# Autodesk Inventor assembly: Segment_Staender_v1
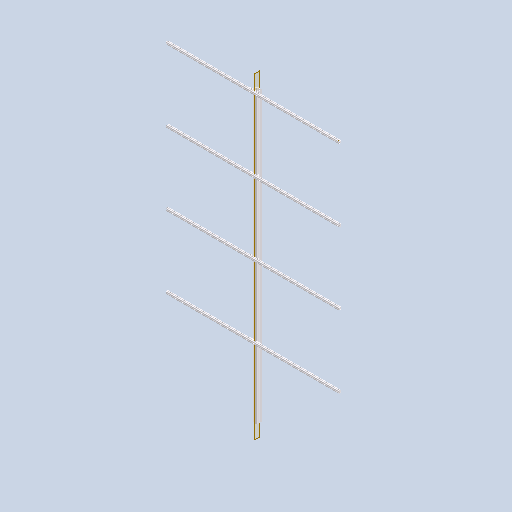
[picture p0: Inventor's stored thumbnail of the model, 512x512]
Saved by Autodesk Inventor 2025.1 (Build 291241000, 241)
## iProperties
Created: 2024-10-13
Part Number: Segment_Staender_v1
Document SubType Name: Assembly
Designer: Kai Altwicker
Author: Kai Altwicker
## Documents named in this file (5)
- C:\Users\tallA\Repos\VolumanXR\hardware-capture\cad\rig_v1\Segment_Staender_v1.iam
- C:\Users\tallA\Repos\VolumanXR\hardware-capture\cad\Library\Profil_5_40x40_2500\Profil_5_40x40_2500\Profil_5_40x40_2500.ipt
- C:\Users\tallA\Repos\VolumanXR\hardware-capture\cad\rig_v1\Profil_5_20x20_1500.ipt
- C:\Users\tallA\Repos\VolumanXR\hardware-capture\cad\Library\Winkelsatz_20x20_einfach\Winkelsatz_20x20_einfach\Winkelsatz_20x20_einfach.ipt
- C:\Users\tallA\Repos\VolumanXR\hardware-capture\cad\dimensions.xlsx
## Components (13 placed, 3 different names)
1. Profil_5_40x40_2500:1 — Passend:4, Fluchtend:7, Passend:5, Fluchtend:11, Passend:7
2. Winkelsatz_20x20_einfach:1 — Passend:5, Passend:6, Fluchtend:10, Fluchtend:12
3. Profil_5_20x20_1500:1 — Passend:4, Fluchtend:7, Passend:6, Fluchtend:10, Fluchtend:11, Passend:8, Passend:9, Passend:10
4. Winkelsatz_20x20_einfach:2 — Passend:7, Passend:8, Fluchtend:12
5. Winkelsatz_20x20_einfach:3
6. Profil_5_20x20_1500:2
7. Winkelsatz_20x20_einfach:4
8. Winkelsatz_20x20_einfach:5
9. Profil_5_20x20_1500:3
10. Winkelsatz_20x20_einfach:6
11. Winkelsatz_20x20_einfach:7
12. Profil_5_20x20_1500:4
13. Winkelsatz_20x20_einfach:8
## Component patterns: (4 elements, first: Winkelsatz_20x20_einfach:1 + Profil_5_20x20_1500:1 + Winkelsatz_20x20_einfach:2)
## Relationships (11: Mate 7, Flush 4)
- Passend:4 [Mate]: Profil_5_40x40_2500:1 ↔ Profil_5_20x20_1500:1
- Fluchtend:7 [Flush]: Profil_5_40x40_2500:1 ↔ Profil_5_20x20_1500:1
- Passend:5 [Mate]: Profil_5_40x40_2500:1 ↔ Winkelsatz_20x20_einfach:1
- Passend:6 [Mate]: Winkelsatz_20x20_einfach:1 ↔ Profil_5_20x20_1500:1
- Fluchtend:10 [Flush]: Winkelsatz_20x20_einfach:1 ↔ Profil_5_20x20_1500:1
- Fluchtend:11 [Flush] (-750 mm): Profil_5_40x40_2500:1 ↔ Profil_5_20x20_1500:1
- Passend:7 [Mate]: Profil_5_40x40_2500:1 ↔ Winkelsatz_20x20_einfach:2
- Passend:8 [Mate]: Profil_5_20x20_1500:1 ↔ Winkelsatz_20x20_einfach:2
- Fluchtend:12 [Flush]: Winkelsatz_20x20_einfach:1 ↔ Winkelsatz_20x20_einfach:2
- Passend:9 [Mate]: Profil_5_20x20_1500:1
- Passend:10 [Mate]: Profil_5_20x20_1500:1
## Named parameters: d_tol = 0.3 mm, d_wand = 1.5 mm, d_traeger = 625 mm, h_profil_20x20 = 20 mm, b_profil_40x40 = 40 mm, b_profil_20x20 = 20 mm, l_profil_20x20 = 1500 mm, l_profil_40x40 = 2500 mm, h_profil_40x40 = 40 mm, D_oct = 3573.03607 mm
